# Autodesk Inventor assembly: Full Assembly v37
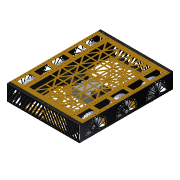
[picture p0: Inventor's stored thumbnail of the model, 180x180]
Saved by Autodesk Inventor 2015 (Build 190159000, 159)
## iProperties
Created: 2014-01-21
Part Number: Full Assembly v37
Document SubType Name: Assembly
Designer: Nick
Mass: 21422.2 g
Surface Area: 59761.8 cm^2
Volume: 9490.75 cm^3
Density: 2.25717 g/cm^3
Author: Nick
## Documents named in this file (18)
- C:\Users\carpe_000\Documents\GitHub\PFPRobot\Mechanical\Drivetrain WIth Cart\Full Assembly v37.iam
- C:\Users\carpe_000\Documents\GitHub\PFPRobot\Mechanical\Drivetrain WIth Cart\Side v9.ipt
- C:\Users\carpe_000\Documents\GitHub\PFPRobot\Mechanical\Drivetrain WIth Cart\Inner v6.ipt
- C:\Users\carpe_000\Documents\GitHub\PFPRobot\Mechanical\Drivetrain WIth Cart\Front v2.ipt
- C:\Users\carpe_000\Documents\GitHub\PFPRobot\Mechanical\Drivetrain WIth Cart\Axle v5.ipt
- C:\Users\carpe_000\Documents\GitHub\PFPRobot\Mechanical\Drivetrain WIth Cart\Cover v3.ipt
- C:\Users\carpe_000\Documents\GitHub\PFPRobot\Mechanical\Drivetrain WIth Cart\Toughbox-mini box.iam
- C:\Users\carpe_000\Documents\GitHub\PFPRobot\Mechanical\Drivetrain WIth Cart\Base v4.ipt
- C:\Users\carpe_000\Documents\GitHub\PFPRobot\Mechanical\Drivetrain WIth Cart\Center Wheel.iam
- C:\Users\carpe_000\Documents\GitHub\PFPRobot\Mechanical\Drivetrain WIth Cart\Outer Wheel.iam
- C:\Users\carpe_000\Documents\GitHub\PFPRobot\Mechanical\Drivetrain WIth Cart\6383K234.ipt
- C:\Users\carpe_000\Documents\GitHub\PFPRobot\Mechanical\Drivetrain WIth Cart\CIM.ipt
- C:\Users\carpe_000\Documents\GitHub\PFPRobot\Mechanical\Drivetrain WIth Cart\Linear Bearing.ipt
- C:\Users\carpe_000\Documents\GitHub\PFPRobot\Mechanical\Drivetrain WIth Cart\Cart Frame.iam
- C:\Users\carpe_000\Documents\GitHub\PFPRobot\Mechanical\Drivetrain WIth Cart\Handle-Cart Link.ipt
- C:\Users\carpe_000\Documents\GitHub\PFPRobot\Mechanical\Drivetrain WIth Cart\Cart Handle.ipt
- C:\Users\carpe_000\Documents\GitHub\PFPRobot\Mechanical\Drivetrain WIth Cart\Cart Handle Pivot.ipt
- C:\Users\carpe_000\Documents\GitHub\PFPRobot\Mechanical\Drivetrain WIth Cart\Battery(Raw).ipt
## Components (35 placed, 17 different names)
1. Side v9:1 — Mate:1, Flush:1, Mate:2, Insert:1, Insert:2, Insert:9, Insert:11, Insert:15, Insert:20, Insert:25, Insert:29
2. Side v9:2 — Insert:3, Insert:4, Insert:14, Insert:21, Insert:28, Insert:30
3. Inner v6:1 — Insert:5, Insert:6, Insert:12, Insert:13, Insert:18, Insert:19, Insert:27, Mate:18, Flush:2, Mate:19, Mate:21, Mate:22, Mate:23, Mate:24, Mate:25, Mate:26
4. Inner v6:2 — Insert:7, Insert:8, Insert:16, Insert:17, Insert:22, Insert:26, Mate:32, Mate:33, Mate:34, Mate:35, Mate:36, Mate:37
5. Front v2:1 — Insert:1, Insert:4, Insert:5, Insert:7
6. Front v2:2 — Insert:2, Insert:3, Insert:6, Insert:8, Flush:3
7. Axle v5:1 — Insert:12
8. Axle v5:2 — Insert:13
9. Axle v5:3 — Insert:11
10. Axle v5:4 — Insert:9
11. Cover v3:1 — Insert:14, Insert:15
12. Toughbox-mini box:1 [sub-assembly] — Insert:18, Insert:19, Mate:41, Mate:42, Mate:44, Mate:45, Mate:46, Mate:50, Mate:51, Mate:52
13. Toughbox-mini box:2 [sub-assembly] — Insert:16, Insert:17, Mate:39, Mate:40, Mate:47, Mate:48, Mate:49, Mate:53, Mate:54, Mate:55
14. Base v4:1 — Insert:20, Insert:21, Insert:22, Mate:43
15. Center Wheel:1 [sub-assembly] — Mate:41, Mate:42, Flush:5
16. Center Wheel:2 [sub-assembly] — Mate:39, Mate:40, Flush:4
17. Outer Wheel:1 [sub-assembly] — Insert:28, Flush:5
18. Outer Wheel:2 [sub-assembly] — Insert:27
19. Outer Wheel:3 [sub-assembly] — Insert:26
20. Outer Wheel:4 [sub-assembly] — Insert:25, Flush:4
21. 6383K234:1 — Insert:30
22. 6383K234:2 — Insert:29
23. CIM:1 — Mate:47, Mate:48, Mate:49
24. CIM:2 — Mate:44, Mate:45, Mate:46
25. Cart Frame:1 [sub-assembly] — Mate:27, Mate:28, Mate:30
26. Cart Handle Pivot:1 — Mate:18, Flush:2, Mate:20, Flush:3
27. Cart Handle:1 — Mate:19, Mate:20, Mate:31, Mate:38
28. Linear Bearing:1 — Mate:24, Mate:25, Mate:26, Mate:28
29. Linear Bearing:2 — Mate:21, Mate:22, Mate:23, Mate:27
30. Linear Bearing:3 — Mate:35, Mate:36, Mate:37
31. Linear Bearing:4 — Mate:32, Mate:33, Mate:34
32. Handle-Cart Link:1 — Mate:30, Mate:31, Mate:38
33. Battery(Raw):1 — Mate:43
34. CIM:3 — Mate:53, Mate:54, Mate:55
35. CIM:4 — Mate:50, Mate:51, Mate:52
## Relationships (71: Mate 39, Insert 27, Flush 5)
- Mate:1: Side v9:1
- Flush:1: Side v9:1
- Mate:2: Side v9:1
- Insert:1: Side v9:1 ↔ Front v2:1
- Insert:2: Side v9:1 ↔ Front v2:2
- Insert:3: Side v9:2 ↔ Front v2:2
- Insert:4: Side v9:2 ↔ Front v2:1
- Insert:5: Inner v6:1 ↔ Front v2:1
- Insert:6: Inner v6:1 ↔ Front v2:2
- Insert:7: Inner v6:2 ↔ Front v2:1
- Insert:8: Inner v6:2 ↔ Front v2:2
- Insert:9: Side v9:1 ↔ Axle v5:4
- Insert:11: Side v9:1 ↔ Axle v5:3
- Insert:12: Inner v6:1 ↔ Axle v5:1
- Insert:13: Inner v6:1 ↔ Axle v5:2
- Insert:14: Side v9:2 ↔ Cover v3:1
- Insert:15: Side v9:1 ↔ Cover v3:1
- Insert:16: Inner v6:2 ↔ Toughbox-mini box:2
- Insert:17: Inner v6:2 ↔ Toughbox-mini box:2
- Insert:18: Inner v6:1 ↔ Toughbox-mini box:1
- Insert:19: Inner v6:1 ↔ Toughbox-mini box:1
- Insert:20: Side v9:1 ↔ Base v4:1
- Insert:21: Side v9:2 ↔ Base v4:1
- Insert:22: Inner v6:2 ↔ Base v4:1
- Insert:25 (43.053 mm): Side v9:1 ↔ Outer Wheel:4
- Insert:26 (43.053 mm): Inner v6:2 ↔ Outer Wheel:3
- Insert:27 (43.053 mm): Inner v6:1 ↔ Outer Wheel:2
- Insert:28 (43.053 mm): Side v9:2 ↔ Outer Wheel:1
- Insert:29: Side v9:1 ↔ 6383K234:2
- Insert:30: Side v9:2 ↔ 6383K234:1
- Mate:18: Inner v6:1 ↔ Cart Handle Pivot:1
- Flush:2: Inner v6:1 ↔ Cart Handle Pivot:1
- Mate:19: Inner v6:1 ↔ Cart Handle:1
- Mate:20: Cart Handle Pivot:1 ↔ Cart Handle:1
- Flush:3 (279.4 mm): Front v2:2 ↔ Cart Handle Pivot:1
- Mate:21: Inner v6:1 ↔ Linear Bearing:2
- Mate:22: Inner v6:1 ↔ Linear Bearing:2
- Mate:23: Inner v6:1 ↔ Linear Bearing:2
- Mate:24: Inner v6:1 ↔ Linear Bearing:1
- Mate:25: Inner v6:1 ↔ Linear Bearing:1
- Mate:26: Inner v6:1 ↔ Linear Bearing:1
- Mate:27: Cart Frame:1 ↔ Linear Bearing:2
- Mate:28: Cart Frame:1 ↔ Linear Bearing:1
- Mate:30: Cart Frame:1 ↔ Handle-Cart Link:1
- Mate:31: Cart Handle:1 ↔ Handle-Cart Link:1
- Mate:32: Inner v6:2 ↔ Linear Bearing:4
- Mate:33: Inner v6:2 ↔ Linear Bearing:4
- Mate:34: Inner v6:2 ↔ Linear Bearing:4
- Mate:35: Inner v6:2 ↔ Linear Bearing:3
- Mate:36: Inner v6:2 ↔ Linear Bearing:3
- Mate:37: Inner v6:2 ↔ Linear Bearing:3
- Mate:38: Cart Handle:1 ↔ Handle-Cart Link:1
- Mate:39: Toughbox-mini box:2 ↔ Center Wheel:2
- Mate:40: Toughbox-mini box:2 ↔ Center Wheel:2
- Flush:4: Center Wheel:2 ↔ Outer Wheel:4
- Mate:41: Toughbox-mini box:1 ↔ Center Wheel:1
- Mate:42: Toughbox-mini box:1 ↔ Center Wheel:1
- Flush:5: Center Wheel:1 ↔ Outer Wheel:1
- Mate:43: Base v4:1 ↔ Battery(Raw):1
- Mate:44: Toughbox-mini box:1 ↔ CIM:2
- Mate:45: Toughbox-mini box:1 ↔ CIM:2
- Mate:46: Toughbox-mini box:1 ↔ CIM:2
- Mate:47: Toughbox-mini box:2 ↔ CIM:1
- Mate:48: Toughbox-mini box:2 ↔ CIM:1
- Mate:49: Toughbox-mini box:2 ↔ CIM:1
- Mate:50: Toughbox-mini box:1 ↔ CIM:4
- Mate:51: Toughbox-mini box:1 ↔ CIM:4
- Mate:52: Toughbox-mini box:1 ↔ CIM:4
- Mate:53: Toughbox-mini box:2 ↔ CIM:3
- Mate:54: Toughbox-mini box:2 ↔ CIM:3
- Mate:55: Toughbox-mini box:2 ↔ CIM:3
